# Autodesk Inventor assembly: Сборка штурвал
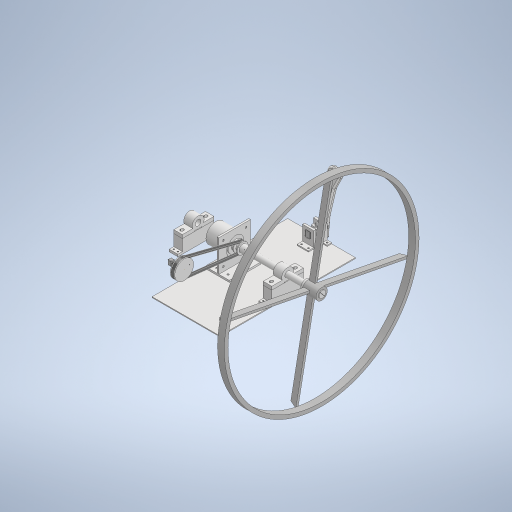
[picture p0: Inventor's stored thumbnail of the model, 512x512]
Saved by Autodesk Inventor 2023 (Build 270158000, 158)
## iProperties
Created: 2022-05-01
Part Number: Сборка штурвал
Document SubType Name: Assembly
Designer: User
Author: User
## Documents named in this file (17)
- D:\Стойка\VR-simulator-3D-models\Механизм\Сборка штурвал.iam
- D:\Стойка\VR-simulator-3D-models\Механизм\Маховик.ipt
- D:\Стойка\VR-simulator-3D-models\Механизм\Вал.ipt
- D:\Стойка\VR-simulator-3D-models\Механизм\Диск (маховик, вал).ipt
- D:\Стойка\VR-simulator-3D-models\Механизм\Стена 16 мм отверстие.ipt
- D:\Стойка\VR-simulator-3D-models\Механизм\Механизм.ipt
- D:\Стойка\VR-simulator-3D-models\Механизм\Подшипник с лапками.ipt
- D:\Стойка\VR-simulator-3D-models\Механизм ручки\Сборка ручка.iam
- D:\Стойка\VR-simulator-3D-models\Механизм\Шкив большой.ipt
- D:\Стойка\VR-simulator-3D-models\Механизм\Подставка подшипника.ipt
- D:\Стойка\VR-simulator-3D-models\Механизм\Шкив малый.ipt
- D:\Стойка\VR-simulator-3D-models\Механизм\Part38.ipt
- D:\Стойка\VR-simulator-3D-models\Механизм\Штурвал.ipt
- D:\Стойка\VR-simulator-3D-models\Механизм\Болт маховика.ipt
- D:\Стойка\VR-simulator-3D-models\Механизм\Двигатель.ipt
- D:\Стойка\VR-simulator-3D-models\Механизм\Сборка штурвал\Мастер проектирования\Передача клиновым ремнем4.iam
- D:\Стойка\VR-simulator-3D-models\Механизм\Кронштейн мотора.ipt
## Components (19 placed, 16 different names)
1. Стена 16 мм отверстие:1 — Заподлицо:1
2. Стена 16 мм отверстие:2 — Заподлицо:1
3. Механизм:1 — Совмещение:18, Заподлицо:2, Совмещение:31, Совмещение:32, Заподлицо:7, Совмещение:40, Совмещение:41, Совмещение:42, Совмещение:70
4. Подшипник с лапками:1 — Цилиндрический:22, Заподлицо:5, Заподлицо:6
5. Подшипник с лапками:2 — Цилиндрический:22, Совмещение:21, Заподлицо:3, Совмещение:33, Заподлицо:4
6. Сборка ручка:1 [sub-assembly] — Совмещение:18, Заподлицо:2, Совмещение:42
7. Вал:1 — Совмещение:21, Совмещение:22, Совмещение:23, Совмещение:24, Совмещение:59, Совмещение:60
8. Диск (маховик, вал):1 — Совмещение:22, Совмещение:23, Совмещение:24, Совмещение:27, С поворотом:2
9. Маховик:1 — Совмещение:27, Совмещение:56, Совмещение:57, С поворотом:2
10. Подставка подшипника:1 — Совмещение:31, Заподлицо:5, Заподлицо:6
11. Подставка подшипника:2 — Совмещение:32, Заподлицо:3, Совмещение:33, Заподлицо:4, Заподлицо:7, Совмещение:40, Совмещение:41
12. Шкив малый:1 — Совмещение:59, Совмещение:60, Совмещение:61, Совмещение:62, Совмещение:68, Заподлицо:8, Совмещение:69
13. Штурвал:1 — Совмещение:54, Совмещение:55, Совмещение:56, Совмещение:57
14. Болт маховика:1 — Совмещение:54, Совмещение:55
15. Двигатель:1 — Совмещение:61, Совмещение:62, Совмещение:71
16. Шкив большой:2 — Совмещение:63, Совмещение:64, Совмещение:66, Заподлицо:8
17. Part38:2 — Совмещение:63, Совмещение:64
18. Передача клиновым ремнем:1 [sub-assembly] — Совмещение:66, Совмещение:68, Совмещение:69
19. Кронштейн мотора:1 — Совмещение:70, Совмещение:71
## Relationships (37: Mate 27, Flush 8, CylindricalJoint 1, RevoluteJoint 1)
- Заподлицо:1 [Flush]: Стена 16 мм отверстие:1 ↔ Стена 16 мм отверстие:2
- Совмещение:18 [Mate]: Механизм:1 ↔ Сборка ручка:1
- Заподлицо:2 [Flush]: Механизм:1 ↔ Сборка ручка:1
- Цилиндрический:22 [CylindricalJoint]: Подшипник с лапками:1 ↔ Подшипник с лапками:2
- Совмещение:21 [Mate]: Подшипник с лапками:2 ↔ Вал:1
- Совмещение:22 [Mate]: Вал:1 ↔ Диск (маховик, вал):1
- Совмещение:23 [Mate]: Вал:1 ↔ Диск (маховик, вал):1
- Совмещение:24 [Mate]: Вал:1 ↔ Диск (маховик, вал):1
- Совмещение:27 [Mate]: Диск (маховик, вал):1 ↔ Маховик:1
- Совмещение:31 [Mate]: Механизм:1 ↔ Подставка подшипника:1
- Совмещение:32 [Mate]: Механизм:1 ↔ Подставка подшипника:2
- Заподлицо:3 [Flush]: Подшипник с лапками:2 ↔ Подставка подшипника:2
- Совмещение:33 [Mate]: Подшипник с лапками:2 ↔ Подставка подшипника:2
- Заподлицо:4 [Flush]: Подшипник с лапками:2 ↔ Подставка подшипника:2
- Заподлицо:5 [Flush]: Подшипник с лапками:1 ↔ Подставка подшипника:1
- Заподлицо:6 [Flush]: Подшипник с лапками:1 ↔ Подставка подшипника:1
- Заподлицо:7 [Flush]: Механизм:1 ↔ Подставка подшипника:2
- Совмещение:40 [Mate]: Механизм:1 ↔ Подставка подшипника:2
- Совмещение:41 [Mate]: Механизм:1 ↔ Подставка подшипника:2
- Совмещение:42 [Mate]: Механизм:1 ↔ Сборка ручка:1
- Совмещение:54 [Mate]: Штурвал:1 ↔ Болт маховика:1
- Совмещение:55 [Mate]: Штурвал:1 ↔ Болт маховика:1
- Совмещение:56 [Mate]: Маховик:1 ↔ Штурвал:1
- Совмещение:57 [Mate]: Маховик:1 ↔ Штурвал:1
- С поворотом:2 [RevoluteJoint]: Диск (маховик, вал):1 ↔ Маховик:1
- Совмещение:59 [Mate]: Вал:1 ↔ Шкив малый:1
- Совмещение:60 [Mate]: Вал:1 ↔ Шкив малый:1
- Совмещение:61 [Mate]: Шкив малый:1 ↔ Двигатель:1
- Совмещение:62 [Mate]: Шкив малый:1 ↔ Двигатель:1
- Совмещение:63 [Mate]: Шкив большой:2 ↔ Part38:2
- Совмещение:64 [Mate]: Шкив большой:2 ↔ Part38:2
- Совмещение:66 [Mate]: Шкив большой:2 ↔ Передача клиновым ремнем:1
- Совмещение:68 [Mate]: Шкив малый:1 ↔ Передача клиновым ремнем:1
- Заподлицо:8 [Flush]: Шкив малый:1 ↔ Шкив большой:2
- Совмещение:69 [Mate]: Шкив малый:1 ↔ Передача клиновым ремнем:1
- Совмещение:70 [Mate]: Механизм:1 ↔ Кронштейн мотора:1
- Совмещение:71 [Mate]: Двигатель:1 ↔ Кронштейн мотора:1
